# Autodesk Inventor assembly: EnsambleCajaControl
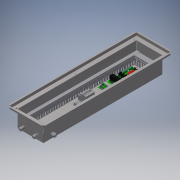
[picture p0: Inventor's stored thumbnail of the model, 180x180]
Saved by Autodesk Inventor 2017 (Build 210142000, 142)
## iProperties
Created: 2021-02-22
Part Number: EnsambleCajaControl
Document SubType Name: Assembly
Designer: USUARIO
Author: USUARIO
## Documents named in this file (10)
- D:\Laboratorio\Modulo Flujo Laminar\2021\JPCFLVMOD-2PM TOUCH Abaco OP202130 #0045884XX\Modelo\EnsambleCajaControl.iam
- D:\Laboratorio\Modulo Flujo Laminar\2021\JPCFLVMOD-2PM TOUCH Abaco OP202130 #0045884XX\Modelo\CAJA CONEXIONES CPM-200-2021.ipt
- D:\Laboratorio\Modulo Flujo Laminar\2021\JPCFLVMOD-2PM TOUCH Abaco OP202130 #0045884XX\Schematic\BoardModuloFlujoLaminar.ipt
- D:\Laboratorio\Modulo Flujo Laminar\2021\JPCFLVMOD-2PM TOUCH Abaco OP202130 #0045884XX\Schematic I2C-RS485\Board_RS485_I2C.ipt
- C:\Modelos 3D y DXF\B1A-NOARK.stp\75856.ipt
- C:\Modelos 3D y DXF\Prensacables\User Library-BUD CABLE GLAND.ipt
- C:\Users\USUARIO\Documents\Inventor\Canaleta 30x60 940mm.iam
- C:\Users\USUARIO\Documents\Inventor\Canaleta 40x60 150mm.iam
- C:\Modelos 3D y DXF\Rele Relpol 2C\PZ8.ipt
- D:\Laboratorio\Modulo Flujo Laminar\2021\JPCFLVMOD-2PM TOUCH Abaco OP202130 #0045884XX\Modelo\Riel120mm.ipt
## Components (15 placed, 9 different names)
1. CAJA CONEXIONES CPM-200-2021:1 — Mate:1, Mate:2, Mate:3, Mate:4, Mate:5, Mate:6, Mate:7, Insert:1, Insert:2, Mate:8, Mate:9, Mate:10, Insert:3, Mate:11, Mate:12, Mate:13, Mate:14, Mate:15, Mate:16, Mate:17, Mate:19, Mate:21, Mate:22, Mate:23, Mate:25, Insert:4
2. BoardModuloFlujoLaminar:1 — Mate:1, Mate:2
3. Board_RS485_I2C:1 — Mate:3, Mate:26
4. 75856:1 — Mate:4, Mate:5
5. User Library-BUD CABLE GLAND:1 — Mate:7, Insert:2
6. User Library-BUD CABLE GLAND:2 — Mate:6, Insert:1
7. 75856:2 — Mate:8, Mate:9, Mate:24
8. User Library-BUD CABLE GLAND:3 — Mate:10, Insert:3
9. Canaleta 30x60 940mm:1 [sub-assembly] — Mate:13, Mate:14, Mate:15, Mate:18, Mate:26
10. Canaleta 30x60 940mm:2 [sub-assembly] — Mate:11, Mate:12, Mate:16, Mate:20
11. Canaleta 40x60 150mm:1 [sub-assembly] — Mate:17, Mate:18, Mate:21
12. Canaleta 40x60 150mm:2 [sub-assembly] — Mate:19, Mate:20, Mate:22
13. PZ8:1 — Mate:23, Mate:24, Flush:1
14. Riel120mm:1 — Mate:25, Flush:1
15. User Library-BUD CABLE GLAND:4 — Insert:4
## Relationships (31: Mate 26, Insert 4, Flush 1)
- Mate:1 (50 mm): CAJA CONEXIONES CPM-200-2021:1 ↔ BoardModuloFlujoLaminar:1
- Mate:2: CAJA CONEXIONES CPM-200-2021:1 ↔ BoardModuloFlujoLaminar:1
- Mate:3 (10 mm): CAJA CONEXIONES CPM-200-2021:1 ↔ Board_RS485_I2C:1
- Mate:4 (3 mm): CAJA CONEXIONES CPM-200-2021:1 ↔ 75856:1
- Mate:5 (60 mm): CAJA CONEXIONES CPM-200-2021:1 ↔ 75856:1
- Mate:6: CAJA CONEXIONES CPM-200-2021:1 ↔ User Library-BUD CABLE GLAND:2
- Mate:7: CAJA CONEXIONES CPM-200-2021:1 ↔ User Library-BUD CABLE GLAND:1
- Insert:1: CAJA CONEXIONES CPM-200-2021:1 ↔ User Library-BUD CABLE GLAND:2
- Insert:2: CAJA CONEXIONES CPM-200-2021:1 ↔ User Library-BUD CABLE GLAND:1
- Mate:8 (3 mm): CAJA CONEXIONES CPM-200-2021:1 ↔ 75856:2
- Mate:9 (60 mm): CAJA CONEXIONES CPM-200-2021:1 ↔ 75856:2
- Mate:10: CAJA CONEXIONES CPM-200-2021:1 ↔ User Library-BUD CABLE GLAND:3
- Insert:3: CAJA CONEXIONES CPM-200-2021:1 ↔ User Library-BUD CABLE GLAND:3
- Mate:11: CAJA CONEXIONES CPM-200-2021:1 ↔ Canaleta 30x60 940mm:2
- Mate:12 (0.5 mm): CAJA CONEXIONES CPM-200-2021:1 ↔ Canaleta 30x60 940mm:2
- Mate:13: CAJA CONEXIONES CPM-200-2021:1 ↔ Canaleta 30x60 940mm:1
- Mate:14 (0.5 mm): CAJA CONEXIONES CPM-200-2021:1 ↔ Canaleta 30x60 940mm:1
- Mate:15 (1 mm): CAJA CONEXIONES CPM-200-2021:1 ↔ Canaleta 30x60 940mm:1
- Mate:16 (1 mm): CAJA CONEXIONES CPM-200-2021:1 ↔ Canaleta 30x60 940mm:2
- Mate:17: CAJA CONEXIONES CPM-200-2021:1 ↔ Canaleta 40x60 150mm:1
- Mate:18 (0.5 mm): Canaleta 30x60 940mm:1 ↔ Canaleta 40x60 150mm:1
- Mate:19: CAJA CONEXIONES CPM-200-2021:1 ↔ Canaleta 40x60 150mm:2
- Mate:20 (0.5 mm): Canaleta 30x60 940mm:2 ↔ Canaleta 40x60 150mm:2
- Mate:21 (30 mm): CAJA CONEXIONES CPM-200-2021:1 ↔ Canaleta 40x60 150mm:1
- Mate:22 (5 mm): CAJA CONEXIONES CPM-200-2021:1 ↔ Canaleta 40x60 150mm:2
- Mate:23: CAJA CONEXIONES CPM-200-2021:1 ↔ PZ8:1
- Mate:24 (2 mm): 75856:2 ↔ PZ8:1
- Mate:25: CAJA CONEXIONES CPM-200-2021:1 ↔ Riel120mm:1
- Flush:1 (-5 mm): PZ8:1 ↔ Riel120mm:1
- Mate:26 (28 mm): Board_RS485_I2C:1 ↔ Canaleta 30x60 940mm:1
- Insert:4: CAJA CONEXIONES CPM-200-2021:1 ↔ User Library-BUD CABLE GLAND:4
